# Autodesk Inventor assembly: assembly roket
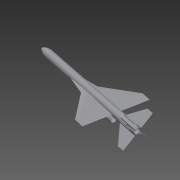
[picture p0: Inventor's stored thumbnail of the model, 180x180]
Saved by Autodesk Inventor 2014 SP1 (Build 180222100, 222)
## iProperties
Created: 2018-05-06
Part Number: assembly roket
Document SubType Name: Assembly
Designer: Dadang
Author: Dadang
## Documents named in this file (6)
- D:\Gambar Inventor\Wahana Roket\assembly roket.iam
- D:\Gambar Inventor\Wahana Roket\Fuselage.ipt
- D:\Gambar Inventor\Wahana Roket\vertikal stab.ipt
- D:\Gambar Inventor\Wahana Roket\EDF Cone.ipt
- D:\Gambar Inventor\Wahana Roket\roket kontruction\wing f16.ipt
- D:\Gambar Inventor\Wahana Roket\roket kontruction\wing f16 kanan.ipt
## Components (8 placed, 5 different names)
1. Fuselage:1 — Mate:25, Mate:26, Mate:27, Mate:34, Mate:35, Mate:36, Mate:40, Mate:41, Mate:42, Mate:43, Mate:44, Mate:45, Mate:46, Mate:47, Mate:48, Mate:49, Mate:50, Mate:51, Mate:52, Mate:53, Mate:54
2. vertikal stab:1 — Mate:25, Mate:26, Mate:27
3. EDF Cone:1 — Mate:34, Mate:35, Mate:36
4. wing f16:1 — Mate:40, Mate:41, Mate:42
5. wing f16 kanan:1 — Mate:43, Mate:44, Mate:45
6. vertikal stab:2 — Mate:51, Mate:52, Mate:54
7. vertikal stab:3 — Mate:49, Mate:50, Mate:53
8. vertikal stab:4 — Mate:46, Mate:47, Mate:48
## Relationships (21: Mate 21)
- Mate:25: Fuselage:1 ↔ vertikal stab:1
- Mate:26: Fuselage:1 ↔ vertikal stab:1
- Mate:27: Fuselage:1 ↔ vertikal stab:1
- Mate:34: Fuselage:1 ↔ EDF Cone:1
- Mate:35: Fuselage:1 ↔ EDF Cone:1
- Mate:36: Fuselage:1 ↔ EDF Cone:1
- Mate:40: Fuselage:1 ↔ wing f16:1
- Mate:41: Fuselage:1 ↔ wing f16:1
- Mate:42: Fuselage:1 ↔ wing f16:1
- Mate:43: Fuselage:1 ↔ wing f16 kanan:1
- Mate:44: Fuselage:1 ↔ wing f16 kanan:1
- Mate:45: Fuselage:1 ↔ wing f16 kanan:1
- Mate:46: Fuselage:1 ↔ vertikal stab:4
- Mate:47: Fuselage:1 ↔ vertikal stab:4
- Mate:48: Fuselage:1 ↔ vertikal stab:4
- Mate:49: Fuselage:1 ↔ vertikal stab:3
- Mate:50: Fuselage:1 ↔ vertikal stab:3
- Mate:51: Fuselage:1 ↔ vertikal stab:2
- Mate:52: Fuselage:1 ↔ vertikal stab:2
- Mate:53: Fuselage:1 ↔ vertikal stab:3
- Mate:54: Fuselage:1 ↔ vertikal stab:2
